# Autodesk Inventor assembly: 6P Sprocket
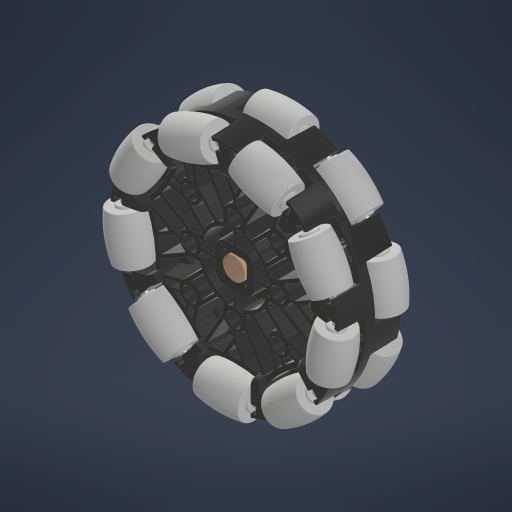
[picture p0: Inventor's stored thumbnail of the model, 512x512]
Saved by Autodesk Inventor 2023 (Build 270158000, 158)
## iProperties
Created: 2022-08-02
Part Number: 6P Sprocket
Document SubType Name: Assembly
Designer: ylu12
Author: ylu12
## Documents named in this file (3)
- D:\GrabCAD\final\VEX-CAD-Inventor-1.4.0\Motion\Wheels\Omni Wheel\2.75 Omni AS, No Insert.iam
- D:\GrabCAD\final\VEX-CAD-Inventor-1.4.0\Motion\Wheels\Reference Files\2.75 Omni Antistatic.ipt
- D:\GrabCAD\final\VEX-CAD-Inventor-1.4.0\Motion\Wheels\Omni Wheel.iam
## Components (1 placed, 1 different names)
1. 2.75 Omni Antistatic
## Relationships (3: Mate 2, Flush 1)
- [Flush]: 2.75 Omni Antistatic
- [Mate]: 2.75 Omni Antistatic
- [Mate]: 2.75 Omni Antistatic
